# Autodesk Inventor assembly: doorLockAssembly_V3
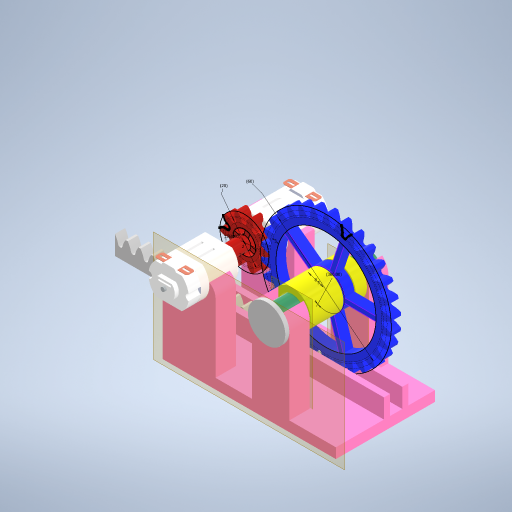
[picture p0: Inventor's stored thumbnail of the model, 512x512]
Saved by Autodesk Inventor 2023 (Build 270158000, 158)
## iProperties
Created: 2022-11-24
Part Number: doorLockAssembly_V3
Document SubType Name: Assembly
Designer: shrey
Author: shrey
## Documents named in this file (11)
- D:\Inventor Projects\Door Lock\V3\doorLockAssembly_V3.iam
- D:\Inventor Projects\Door Lock\V3\doorLockAssembly_V3\Design Accelerator\Spur Gears2.iam
- D:\Inventor Projects\Door Lock\V3\gear_V3.ipt
- D:\Inventor Projects\Door Lock\V3\pinion_V3.ipt
- D:\Inventor Projects\Door Lock\motor.ipt
- D:\Inventor Projects\Door Lock\V3\tempMotorHolder_V3.ipt
- D:\Inventor Projects\Door Lock\V3\pin_V3.ipt
- D:\Inventor Projects\Door Lock\V3\spacerA_V3.ipt
- D:\Inventor Projects\Door Lock\V3\spacerB_V3.ipt
- D:\Inventor Projects\Door Lock\V3\rack_V3.ipt
- D:\Inventor Projects\Door Lock\V3\pinEndCap_V3.ipt
## Components (11 placed, 10 different names)
1. Reference Spur Gears:1 [sub-assembly] — Mate:5, Mate:6, Mate:7
2. gear_V3:1 — Mate:3, Mate:4, Tangent:1, Rotation:1, Mate:11, Mate:12, Mate:13, Flush:10, Rotation/Translation:1, Mate:15
3. pinion_V3:1 — Mate:1, Mate:2, Tangent:1, Rotation:1, Mate:9, Flush:4
4. motor:1 — Flush:1, Mate:8, Flush:2
5. motor:2 — Mate:9, Mate:10, Flush:3, Flush:5
6. tempMotorHolder_V3:1 — Flush:4, Flush:5, Flush:6, Flush:7, Flush:8, Flush:9, Mate:14, Mate:16
7. pin_V3:1 — Flush:6, Mate:11, Flush:7, Mate:12, Flush:11, Mate:15, Mate:17
8. spacerA_V3:1 — Flush:8
9. spacerB_V3:1 — Flush:9, Mate:13
10. rack_V3:1 — Mate:14, Flush:10, Rotation/Translation:1
11. pinEndCap_V3:1 — Flush:11, Mate:16, Mate:17
## Relationships (31: Mate 17, Flush 11, Tangent 1, RelateRotation 1, RelateRotateTranslate 1)
- Mate:1: pinion_V3:1
- Mate:2: pinion_V3:1
- Mate:3: gear_V3:1
- Mate:4: gear_V3:1
- Tangent:1: gear_V3:1 ↔ pinion_V3:1
- Mate:5: Reference Spur Gears:1
- Mate:6: Reference Spur Gears:1
- Mate:7: Reference Spur Gears:1
- Flush:1: motor:1
- Mate:8: motor:1
- Flush:2: motor:1
- Rotation:1 [RelateRotation] (0.333 ul): gear_V3:1 ↔ pinion_V3:1
- Mate:9: pinion_V3:1 ↔ motor:2
- Mate:10: motor:2
- Flush:3: motor:2
- Flush:4 (-7.78 mm): pinion_V3:1 ↔ tempMotorHolder_V3:1
- Flush:5 (-5 mm): motor:2 ↔ tempMotorHolder_V3:1
- Flush:6: tempMotorHolder_V3:1 ↔ pin_V3:1
- Mate:11: gear_V3:1 ↔ pin_V3:1
- Flush:7: tempMotorHolder_V3:1 ↔ pin_V3:1
- Flush:8 (0.5 mm): tempMotorHolder_V3:1 ↔ spacerA_V3:1
- Flush:9 (0.5 mm): tempMotorHolder_V3:1 ↔ spacerB_V3:1
- Mate:12: gear_V3:1 ↔ pin_V3:1
- Mate:13: gear_V3:1 ↔ spacerB_V3:1
- Mate:14: tempMotorHolder_V3:1 ↔ rack_V3:1
- Flush:10: gear_V3:1 ↔ rack_V3:1
- Rotation/Translation:1 [RelateRotateTranslate] (188.4956 mm): gear_V3:1 ↔ rack_V3:1
- Flush:11: pin_V3:1 ↔ pinEndCap_V3:1
- Mate:15: gear_V3:1 ↔ pin_V3:1
- Mate:16: tempMotorHolder_V3:1 ↔ pinEndCap_V3:1
- Mate:17: pin_V3:1 ↔ pinEndCap_V3:1
